# Autodesk Inventor assembly: 滑台
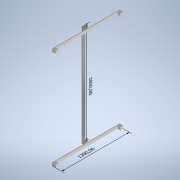
[picture p0: Inventor's stored thumbnail of the model, 180x180]
Saved by Autodesk Inventor 2020 (Build 240168000, 168)
## iProperties
Created: 2021-04-05
Part Number: 滑台
Document SubType Name: Assembly
Designer: 70929
Author: 70929
## Documents named in this file (3)
- D:\大创\图书整理机器人\建模\部件\滑台.iam
- D:\大创\图书整理机器人\建模\竖直滑台.ipt
- D:\大创\图书整理机器人\建模\水平滑台.ipt
## Components (3 placed, 2 different names)
1. 竖直滑台:1 — 表面齐平:1, 配合:1, 配合:2
2. 竖直滑台:2 — 表面齐平:1, 配合:1, 滑块:1
3. 水平滑台:1 — 滑块:1, 配合:2
## Relationships (4: Mate 2, Flush 1, TranslationJoint 1)
- 表面齐平:1 [Flush]: 竖直滑台:1 ↔ 竖直滑台:2
- 配合:1 [Mate]: 竖直滑台:1 ↔ 竖直滑台:2
- 滑块:1 [TranslationJoint]: 竖直滑台:2 ↔ 水平滑台:1
- 配合:2 [Mate]: 竖直滑台:1 ↔ 水平滑台:1
